# Autodesk Inventor assembly: MotorArm
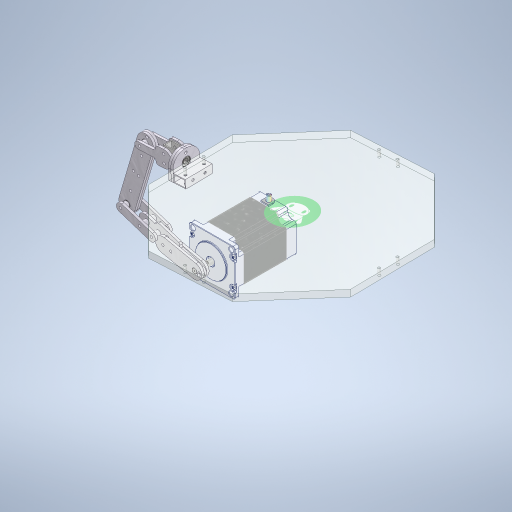
[picture p0: Inventor's stored thumbnail of the model, 512x512]
Saved by Autodesk Inventor 2023 (Build 270158000, 158)
## iProperties
Created: 2024-02-07
Part Number: MotorArm
Document SubType Name: Assembly
Designer: victo
Author: victo
## Documents named in this file (15)
- C:\Users\victo\Documents\ball-balancing-digital-twin\Mechanics\CAD\MotorArm.iam
- C:\Users\victo\Documents\ball-balancing-digital-twin\Mechanics\CAD\Step Motor Nema AK23 - 15kg.ipt
- C:\Users\victo\Documents\ball-balancing-digital-twin\Mechanics\CAD\motorAxis.ipt
- C:\Users\victo\Documents\ball-balancing-digital-twin\Mechanics\CAD\Arm1.ipt
- C:\Users\victo\Documents\ball-balancing-digital-twin\Mechanics\CAD\Arm2.ipt
- C:\Users\victo\Documents\ball-balancing-digital-twin\Mechanics\CAD\Arm3.ipt
- C:\Users\victo\Documents\ball-balancing-digital-twin\Mechanics\CAD\spacer.ipt
- C:\Users\victo\Documents\ball-balancing-digital-twin\Mechanics\CAD\bearing 1.ipt
- C:\Users\victo\Documents\ball-balancing-digital-twin\Mechanics\CAD\Arm4.ipt
- C:\Users\victo\Documents\ball-balancing-digital-twin\Mechanics\CAD\spacer2.ipt
- C:\Users\victo\Documents\ball-balancing-digital-twin\Mechanics\CAD\Arm5.ipt
- C:\Users\victo\Documents\ball-balancing-digital-twin\Mechanics\CAD\profile1.ipt
- C:\Users\victo\Documents\ball-balancing-digital-twin\Mechanics\CAD\Arm6.ipt
- C:\Users\victo\Documents\ball-balancing-digital-twin\Mechanics\CAD\profile2.ipt
- C:\Users\victo\Documents\ball-balancing-digital-twin\Mechanics\CAD\Plate_Acrylic.ipt
## Components (27 placed, 14 different names)
1. Step Motor Nema AK23 - 15kg:1 — Rotational:1
2. motorAxis:1 — Mate:2, Angle:1, Mate:3, Angle:2, Mate:5, Angle:3, Flush:2, Rotational:1
3. Arm1:1 — Mate:2, Angle:1, Mate:4, Mate:6, Mate:7, Mate:8, Mate:9, Mate:10, Mate:11, Mate:12, Mate:13, Mate:14
4. Arm2:1 — Mate:3, Angle:2, Mate:4, Flush:2
5. Arm2:2 — Mate:5, Angle:3, Mate:6
6. spacer:1 — Mate:7, Mate:10, Mate:18, Mate:19
7. spacer:2 — Mate:8, Mate:9, Mate:20
8. spacer:3 — Mate:12, Mate:14, Mate:17
9. spacer:4 — Mate:11, Mate:13, Mate:15, Mate:16
10. Arm3:2 — Mate:15, Mate:16, Mate:17, Mate:21, Mate:29, Mate:31
11. Arm3:3 — Mate:18, Mate:19, Mate:20, Mate:30, Mate:32
12. bearing 1:1 — Mate:21, Mate:22, Mate:23, Mate:24, Mate:28, Mate:33
13. Arm4:1 — Mate:22, Mate:23, Mate:25
14. Arm4:2 — Mate:24, Mate:26, Mate:27, Mate:28
15. bearing 1:2 — Mate:25, Mate:26, Mate:27, Mate:34, Mate:35, Mate:36, Mate:37, Mate:38, Mate:39
16. spacer2:1 — Mate:29, Mate:31, Mate:33
17. spacer2:2 — Mate:30, Mate:32
18. Arm5:1 — Mate:34, Mate:41, Mate:42, Mate:43
19. Arm5:2 — Mate:35, Mate:40, Mate:44, Mate:45, Mate:46
20. spacer2:3 — Mate:37, Mate:38, Mate:41
21. spacer2:4 — Mate:36, Mate:39, Mate:40
22. profile1:1 — Mate:42, Mate:43, Mate:44, Mate:45, Mate:46, Mate:47, Mate:53
23. Arm6:1 — Mate:47, Mate:48, Mate:49, Mate:51, Mate:52, Mate:53
24. bearing 1:3 — Mate:48, Mate:49, Mate:50
25. Arm6:2 — Mate:50, Mate:51, Mate:52, Mate:54, Mate:55, Mate:56
26. profile2:1 — Mate:54, Mate:55, Mate:56, Mate:57, Mate:58, Mate:59
27. Plate_Acrylic:1 — Mate:57, Mate:58, Mate:59
## Relationships (63: Mate 58, Angle 3, Flush 1, RevoluteJoint 1)
- Mate:2: motorAxis:1 ↔ Arm1:1
- Angle:1 (180 deg): motorAxis:1 ↔ Arm1:1
- Mate:3: motorAxis:1 ↔ Arm2:1
- Angle:2 (180 deg): motorAxis:1 ↔ Arm2:1
- Mate:4: Arm1:1 ↔ Arm2:1
- Mate:5: motorAxis:1 ↔ Arm2:2
- Angle:3 (180 deg): motorAxis:1 ↔ Arm2:2
- Mate:6: Arm1:1 ↔ Arm2:2
- Mate:7: Arm1:1 ↔ spacer:1
- Mate:8: Arm1:1 ↔ spacer:2
- Mate:9: Arm1:1 ↔ spacer:2
- Mate:10: Arm1:1 ↔ spacer:1
- Flush:2: motorAxis:1 ↔ Arm2:1
- Mate:11: Arm1:1 ↔ spacer:4
- Mate:12: Arm1:1 ↔ spacer:3
- Mate:13: Arm1:1 ↔ spacer:4
- Mate:14: Arm1:1 ↔ spacer:3
- Mate:15: spacer:4 ↔ Arm3:2
- Mate:16: spacer:4 ↔ Arm3:2
- Mate:17: spacer:3 ↔ Arm3:2
- Mate:18: spacer:1 ↔ Arm3:3
- Mate:19: spacer:1 ↔ Arm3:3
- Mate:20: spacer:2 ↔ Arm3:3
- Mate:21: Arm3:2 ↔ bearing 1:1
- Mate:22: bearing 1:1 ↔ Arm4:1
- Mate:23: bearing 1:1 ↔ Arm4:1
- Mate:24: bearing 1:1 ↔ Arm4:2
- Mate:25: Arm4:1 ↔ bearing 1:2
- Mate:26: Arm4:2 ↔ bearing 1:2
- Mate:27: Arm4:2 ↔ bearing 1:2
- Mate:28: bearing 1:1 ↔ Arm4:2
- Mate:29: Arm3:2 ↔ spacer2:1
- Mate:30: Arm3:3 ↔ spacer2:2
- Mate:31: Arm3:2 ↔ spacer2:1
- Mate:32: Arm3:3 ↔ spacer2:2
- Mate:33: bearing 1:1 ↔ spacer2:1
- Rotational:1 [RevoluteJoint]: Step Motor Nema AK23 - 15kg:1 ↔ motorAxis:1
- Mate:34: bearing 1:2 ↔ Arm5:1
- Mate:35: bearing 1:2 ↔ Arm5:2
- Mate:36: bearing 1:2 ↔ spacer2:4
- Mate:37: bearing 1:2 ↔ spacer2:3
- Mate:38: bearing 1:2 ↔ spacer2:3
- Mate:39: bearing 1:2 ↔ spacer2:4
- Mate:40: Arm5:2 ↔ spacer2:4
- Mate:41: Arm5:1 ↔ spacer2:3
- Mate:42: Arm5:1 ↔ profile1:1
- Mate:43: Arm5:1 ↔ profile1:1
- Mate:44 (2 mm): Arm5:2 ↔ profile1:1
- Mate:45: Arm5:2 ↔ profile1:1
- Mate:46: Arm5:2 ↔ profile1:1
- Mate:47: profile1:1 ↔ Arm6:1
- Mate:48: Arm6:1 ↔ bearing 1:3
- Mate:49: Arm6:1 ↔ bearing 1:3
- Mate:50: bearing 1:3 ↔ Arm6:2
- Mate:51: Arm6:1 ↔ Arm6:2
- Mate:52: Arm6:1 ↔ Arm6:2
- Mate:53 (2 mm): profile1:1 ↔ Arm6:1
- Mate:54: Arm6:2 ↔ profile2:1
- Mate:55: Arm6:2 ↔ profile2:1
- Mate:56: Arm6:2 ↔ profile2:1
- Mate:57: profile2:1 ↔ Plate_Acrylic:1
- Mate:58: profile2:1 ↔ Plate_Acrylic:1
- Mate:59: profile2:1 ↔ Plate_Acrylic:1
